# Autodesk Inventor assembly: Effector_ZProbe
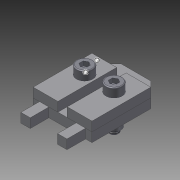
[picture p0: Inventor's stored thumbnail of the model, 180x180]
Saved by Autodesk Inventor 2014 (Build 180170000, 170)
## iProperties
Created: 2014-08-28
Part Number: Effector_ZProbe
Document SubType Name: Assembly
Designer: ThatOtherGuy
Author: ThatOtherGuy
## Documents named in this file (5)
- C:\Users\ThatOtherGuy\Documents\Inventor\KosselCNC1515\Effector\Effector_ZProbe.iam
- C:\Users\ThatOtherGuy\Documents\Inventor\KosselCNC1515\Effector\Effector_ZProbe_A.ipt
- C:\Users\ThatOtherGuy\Documents\Inventor\KosselCNC1515\Effector\Effector_ZProbe_B.ipt
- C:\Users\ThatOtherGuy\Documents\Inventor\Content Center Files\R2014\en-US\ISO 10511\ISO 10511 - M3.ipt
- C:\Users\ThatOtherGuy\Documents\Inventor\Content Center Files\R2014\en-US\ANSI B18.3.1M(1)\ANSI B18.3.1M - M3x0.5 x 12(2).ipt
## Components (7 placed, 4 different names)
1. Effector_ZProbe_A:1 — Mate:1, Mate:2, Mate:3, Mate:4, Flush:1, Flush:2, Insert:3, Insert:4
2. Effector_ZProbe_B:1 — Mate:1, Mate:2, Flush:2, Insert:1
3. Effector_ZProbe_B:2 — Mate:3, Mate:4, Flush:1, Insert:2
4. Broached Socket Head Cap Screw - Metric M3x0.5 x 12:1 — Insert:1
5. Broached Socket Head Cap Screw - Metric M3x0.5 x 12:2 — Insert:2
6. DIN EN ISO 10511 M3:1 — Insert:3
7. DIN EN ISO 10511 M3:2 — Insert:4
## Relationships (10: Mate 4, Insert 4, Flush 2)
- Mate:1: Effector_ZProbe_A:1 ↔ Effector_ZProbe_B:1
- Mate:2: Effector_ZProbe_A:1 ↔ Effector_ZProbe_B:1
- Mate:3: Effector_ZProbe_A:1 ↔ Effector_ZProbe_B:2
- Mate:4: Effector_ZProbe_A:1 ↔ Effector_ZProbe_B:2
- Flush:1: Effector_ZProbe_A:1 ↔ Effector_ZProbe_B:2
- Flush:2: Effector_ZProbe_A:1 ↔ Effector_ZProbe_B:1
- Insert:1: Effector_ZProbe_B:1 ↔ Broached Socket Head Cap Screw - Metric M3x0.5 x 12:1
- Insert:2: Effector_ZProbe_B:2 ↔ Broached Socket Head Cap Screw - Metric M3x0.5 x 12:2
- Insert:3: Effector_ZProbe_A:1 ↔ DIN EN ISO 10511 M3:1
- Insert:4: Effector_ZProbe_A:1 ↔ DIN EN ISO 10511 M3:2
